# Autodesk Inventor assembly: Cockpit_
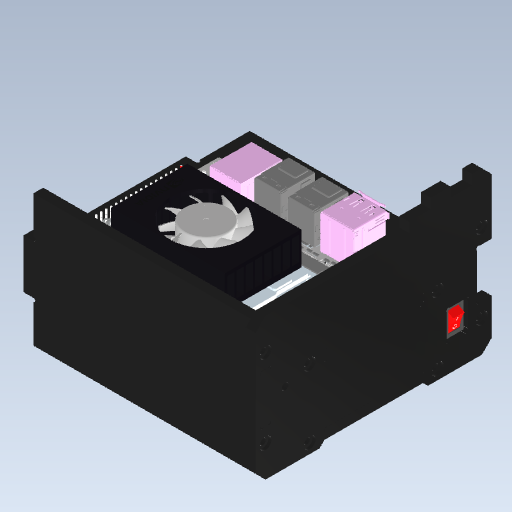
[picture p0: Inventor's stored thumbnail of the model, 512x512]
Saved by Autodesk Inventor 2020.4 (Build 244396000, 396)
## iProperties
Created: 2022-01-06
Part Number: Cockpit_
Document SubType Name: Assembly
Designer: Masato Kubotera
Author: Masato Kubotera
## Documents named in this file (7)
- C:\Users\Masato\Documents\Inventor\CIT Brains_Inventor\OpenPlatform_ver3_0 - ve4_1 branch\UpperBody\Cockpit\Cockpit_.iam
- C:\Users\Masato\Documents\Inventor\CIT Brains_Inventor\OpenPlatform_ver3_0 - ve4_1 branch\UpperBody\Cockpit\Cockpit_side_frame.ipt
- C:\Users\Masato\Documents\Inventor\CIT Brains_Inventor\OpenPlatform_ver3_0 - ve4_1 branch\UpperBody\Cockpit\Cockpit_front_frame.ipt
- C:\Users\Masato\Documents\Inventor\CIT Brains_Inventor\OpenPlatform_ver3_0 - ve4_1 branch\Ready_Made\Jetson_Xavier_NX_DevKit_without_Wi-FiAntennas\Jetson_Xavier_NX_DevKit.iam
- C:\Users\Masato\Documents\Inventor\CIT Brains_Inventor\OpenPlatform_ver3_0 - ve4_1 branch\UpperBody\Cockpit\Cockpit_bottom_frame.ipt
- C:\Users\Masato\Documents\Inventor\CIT Brains_Inventor\OpenPlatform_ver3_0 - ve4_1 branch\UpperBody\Cockpit\Cockpit_middle_frame.ipt
- C:\Users\Masato\Documents\Inventor\CIT Brains_Inventor\OpenPlatform_ver3_0 - ve4_1 branch\Ready_Made\KCD11-A-101011BB.ipt
## Components (6 placed, 6 different names)
1. Cockpit_side_frame:1 — 挿入:1, 挿入:2, 挿入:3, 挿入:4, 挿入:5, 挿入:6, フラッシュ:1, メイト:1, フラッシュ:2, メイト:2, メイト:3, メイト:4
2. Cockpit_front_frame:1 — 挿入:1, 挿入:2
3. Jetson_Xavier_NX_DevKit:1 [sub-assembly] — 挿入:7, 挿入:8
4. Cockpit_bottom_frame:1 — 挿入:3, 挿入:4
5. Cockpit_middle_frame:1 — 挿入:5, 挿入:6, 挿入:7, 挿入:8
6. KCD11-A-101011BB:1 — メイト:2, メイト:3, メイト:4
## Relationships (14: Insert 8, Mate 4, Flush 2)
- 挿入:1 [Insert]: Cockpit_side_frame:1 ↔ Cockpit_front_frame:1
- 挿入:2 [Insert]: Cockpit_side_frame:1 ↔ Cockpit_front_frame:1
- 挿入:3 [Insert]: Cockpit_side_frame:1 ↔ Cockpit_bottom_frame:1
- 挿入:4 [Insert]: Cockpit_side_frame:1 ↔ Cockpit_bottom_frame:1
- 挿入:5 [Insert]: Cockpit_side_frame:1 ↔ Cockpit_middle_frame:1
- 挿入:6 [Insert]: Cockpit_side_frame:1 ↔ Cockpit_middle_frame:1
- 挿入:7 [Insert]: Jetson_Xavier_NX_DevKit:1 ↔ Cockpit_middle_frame:1
- 挿入:8 [Insert]: Jetson_Xavier_NX_DevKit:1 ↔ Cockpit_middle_frame:1
- フラッシュ:1 [Flush]: Cockpit_side_frame:1
- メイト:1 [Mate]: Cockpit_side_frame:1
- フラッシュ:2 [Flush]: Cockpit_side_frame:1
- メイト:2 [Mate] (0.05 mm): Cockpit_side_frame:1 ↔ KCD11-A-101011BB:1
- メイト:3 [Mate] (0.05 mm): Cockpit_side_frame:1 ↔ KCD11-A-101011BB:1
- メイト:4 [Mate]: Cockpit_side_frame:1 ↔ KCD11-A-101011BB:1
